# Autodesk Inventor assembly: Shooter
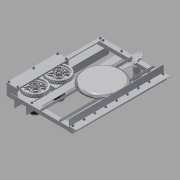
[picture p0: Inventor's stored thumbnail of the model, 180x180]
Saved by Autodesk Inventor 2013 (Build 170138000, 138)
## iProperties
Created: 2013-01-27
Part Number: Shooter
Document SubType Name: Assembly
Designer: Naphat
Author: Naphat
## Documents named in this file (22)
- C:\Autodesk\gruntmaster6000-cad\Shooter6000-cad\Shooter\Shooter.iam
- C:\Autodesk\gruntmaster6000-cad\Shooter6000-cad\Shooter\Basic Wheel\Shooter Basic Design.iam
- C:\Autodesk\gruntmaster6000-cad\Shooter6000-cad\Shooter\26in Angle Channel.ipt
- C:\Autodesk\gruntmaster6000-cad\Shooter6000-cad\Shooter\26in mini C-Channel (rail).ipt
- C:\Autodesk\gruntmaster6000-cad\Shooter6000-cad\Shooter\26in C-Channel (TopPlate Supports).ipt
- C:\Autodesk\gruntmaster6000-cad\Shooter6000-cad\Shooter\3in C-Channel (TopPlate Supports).ipt
- C:\Autodesk\gruntmaster6000-cad\Shooter6000-cad\Shooter\Top Plate.ipt
- C:\Users\Naphat\Documents\Inventor\Content Center Files\R2013\en-US\ANSI B18.3(05)\ANSI B18.3 - 1_4-20 UNC - 1(31).ipt
- C:\Users\Naphat\Documents\Inventor\Content Center Files\R2013\en-US\ASTM F436(1)\ASTM F436 - 1_4(1).ipt
- C:\Users\Naphat\Documents\Inventor\Content Center Files\R2013\en-US\IFI 100 107(2)\IFI 100_107 - 1_4 - 20 Metal Type.ipt
- C:\Autodesk\gruntmaster6000-cad\Shooter6000-cad\Shooter\18in C-Channel Front.ipt
- C:\Autodesk\gruntmaster6000-cad\Shooter6000-cad\Shooter\18in C-Channel Rear.ipt
- C:\Users\Naphat\Documents\Inventor\Content Center Files\R2013\en-US\ANSI B18.3(05)\ANSI B18.3 - 1_4-20 UNC - 1.75(31).ipt
- C:\Autodesk\gruntmaster6000-cad\Shooter6000-cad\Shooter\26in Angle Channel CIM Mount Left.ipt
- C:\Autodesk\gruntmaster6000-cad\Shooter6000-cad\Shooter\26in Angle Channel CIM Mount Right.ipt
- C:\Autodesk\gruntmaster6000-cad\Shooter6000-cad\Shooter\26in C-Channel Left.ipt
- C:\Autodesk\gruntmaster6000-cad\Shooter6000-cad\Shooter\26in C-Channel Right.ipt
- C:\Autodesk\gruntmaster6000-cad\Shooter6000-cad\Shooter\3in C-Channel (TopPlate Supports Rear).ipt
- C:\Autodesk\gruntmaster6000-cad\Shooter6000-cad\Shooter\Motors\CIM Case\CIM Mount Bolt.ipt
- C:\Autodesk\gruntmaster6000-cad\Shooter6000-cad\Shooter\Firing Pin\Firing Pin.iam
- C:\Autodesk\gruntmaster6000-cad\Shooter6000-cad\Shooter\Frisbee.ipt
- C:\Autodesk\gruntmaster6000-cad\Shooter6000-cad\Imported Components\PG27\PG27.ipt
## Components (98 placed, 21 different names)
1. Shooter Basic Design:1 [sub-assembly] — Flush:7, Mate:11, Mate:13, Mate:16, Flush:10, Mate:19, Mate:188
2. Shooter Basic Design:2 [sub-assembly] — Flush:7, Mate:15, Mate:16, Flush:10, Mate:17, Mate:187
3. 26in C-Channel Right:1 — Flush:3, Mate:1, Mate:2, Mate:5, Mate:7, Flush:5, Mate:27, Flush:15, Mate:104, Mate:107, Flush:19, Mate:149, Mate:156, Mate:157, Mate:158
4. 18in C-Channel Rear — Flush:3, Mate:1, Mate:2, Flush:4, Mate:3, Mate:4, Flush:9, Mate:18, Flush:11, Mate:82, Mate:92, Mate:93, Mate:105, Mate:106, Mate:108, Mate:109, Mate:207, Mate:208, Mate:212
5. 18in C-Channel Front — Mate:5, Mate:6, Mate:7, Flush:5, Mate:13, Mate:20, Flush:12, Mate:23, Flush:13, Mate:24, Flush:14, Mate:74, Mate:98, Mate:99, Mate:123, Mate:124, Mate:126, Mate:127, Mate:129, Mate:138
6. 26in C-Channel Left:1 — Flush:4, Mate:3, Mate:4, Mate:6, Mate:8, Mate:9, Mate:75, Mate:76, Mate:77, Mate:78, Mate:79, Mate:80, Mate:81
7. 26in Angle Channel:1 — Mate:8, Mate:9, Flush:9, Mate:11, Mate:15, Mate:25, Mate:36, Mate:38, Mate:39, Mate:40, Mate:41, Mate:42, Mate:43, Mate:44, Mate:45, Mate:46, Mate:47, Mate:48, Mate:49, Mate:50, Mate:51, Mate:52, Mate:53, Mate:54, Mate:55, Mate:56, Mate:57, Mate:58, Mate:59, Mate:60, Mate:61, Mate:62, Mate:63
8. 26in Angle Channel CIM Mount Right:1 — Mate:17, Mate:18, Flush:11, Mate:117, Mate:118, Mate:134, Mate:137, Mate:187, Mate:188, Mate:189, Mate:190, Mate:191, Mate:192, Mate:193, Mate:194, Mate:195, Mate:196
9. 26in Angle Channel CIM Mount Left:3 — Mate:19, Mate:20, Flush:12, Mate:96, Mate:102, Mate:116, Mate:140
10. 26in mini C-Channel (rail):1 — Mate:23, Flush:13, Mate:26, Mate:206
11. 26in mini C-Channel (rail):2 — Mate:24, Flush:14, Mate:25, Mate:26
12. 26in C-Channel (TopPlate Supports):1 — Mate:27, Flush:15, Mate:28, Mate:29, Mate:30, Mate:31, Mate:33, Mate:34, Flush:19, Mate:125, Mate:144, Mate:145, Mate:146, Mate:147, Mate:148, Mate:180, Mate:181, Mate:201, Mate:203
13. 3in C-Channel (TopPlate Supports):1 — Mate:28, Mate:29, Mate:30, Flush:17, Mate:35, Flush:18, Mate:162, Mate:179
14. 3in C-Channel (TopPlate Supports Rear):1 — Mate:31, Mate:33, Mate:34, Mate:182
15. Top Plate:1 — Flush:17, Mate:35, Flush:18, Mate:163, Mate:164, Mate:165, Mate:166, Mate:167, Mate:168, Mate:169, Mate:170, Mate:197, Mate:198, Mate:199
16. CIM Mount Bolt:1 — Mate:192, Mate:196
17. CIM Mount Bolt:2 — Mate:191, Mate:195
18. CIM Mount Bolt:3 — Mate:189, Mate:193
19. CIM Mount Bolt:4 — Mate:190, Mate:194
20. Firing Pin:1 [sub-assembly] — Mate:207, Mate:208, Mate:210, Mate:211
21. Frisbee:1 — Mate:206
22. PG27:1 — Mate:210, Mate:211, Mate:212
23. Hexagon Socket Head Cap Screw - Inch 1/4 - 20 UNC - 1:1 — Mate:36, Mate:72, Mate:91
24. Hexagon Socket Head Cap Screw - Inch 1/4 - 20 UNC - 1:3 — Mate:39, Mate:70, Mate:89
25. Hexagon Socket Head Cap Screw - Inch 1/4 - 20 UNC - 1:4 — Mate:38, Mate:71, Mate:90
26. Hexagon Socket Head Cap Screw - Inch 1/4 - 20 UNC - 1:6 — Mate:199, Mate:200, Mate:202, Mate:204
27. Hexagon Socket Head Cap Screw - Inch 1/4 - 20 UNC - 1:9 — Mate:151, Mate:154, Mate:160
28. Hexagon Socket Head Cap Screw - Inch 1/4 - 20 UNC - 1:10 — Mate:43, Mate:66, Mate:85
29. Hexagon Socket Head Cap Screw - Inch 1/4 - 20 UNC - 1:11 — Mate:40, Mate:69, Mate:88
30. Hexagon Socket Head Cap Screw - Inch 1/4 - 20 UNC - 1:12 — Mate:163, Mate:171, Mate:177, Mate:186
31. Hexagon Socket Head Cap Screw - Inch 1/4 - 20 UNC - 1:14 — Mate:42, Mate:67, Mate:86
32. Hexagon Socket Head Cap Screw - Inch 1/4 - 20 UNC - 1:15 — Mate:173, Mate:176, Mate:184
33. Hexagon Socket Head Cap Screw - Inch 1/4 - 20 UNC - 1:16 — Mate:44, Mate:65, Mate:84
34. Hexagon Socket Head Cap Screw - Inch 1/4 - 20 UNC - 1:17 — Mate:150, Mate:153, Mate:159
35. Hexagon Socket Head Cap Screw - Inch 1/4 - 20 UNC - 1:18 — Mate:45, Mate:64, Mate:83
36. Hexagon Socket Head Cap Screw - Inch 1/4 - 20 UNC - 1:19 — Mate:174, Mate:175, Mate:183
37. Hexagon Socket Head Cap Screw - Inch 1/4 - 20 UNC - 1:22 — Mate:41, Mate:68, Mate:87
38. Hexagon Socket Head Cap Screw - Inch 1/4 - 20 UNC - 1:23 — Mate:152, Mate:155, Mate:161
39. Hexagon Socket Head Cap Screw - Inch 1/4 - 20 UNC - 1:24 — Mate:172, Mate:178, Mate:185
40. Prevailing Torque Type Hex Nut - Inch (IFI) 1/4 - 20 Metal Type:1 — Mate:117, Mate:120
41. Prevailing Torque Type Hex Nut - Inch (IFI) 1/4 - 20 Metal Type:2 — Mate:78, Mate:87
42. Prevailing Torque Type Hex Nut - Inch (IFI) 1/4 - 20 Metal Type:3 — Mate:180, Mate:185
43. Prevailing Torque Type Hex Nut - Inch (IFI) 1/4 - 20 Metal Type:4 — Mate:102, Mate:103
44. Prevailing Torque Type Hex Nut - Inch (IFI) 1/4 - 20 Metal Type:5 — Mate:179, Mate:186
45. Prevailing Torque Type Hex Nut - Inch (IFI) 1/4 - 20 Metal Type:8 — Mate:80, Mate:85
46. Prevailing Torque Type Hex Nut - Inch (IFI) 1/4 - 20 Metal Type:9 — Mate:77, Mate:88
47. Prevailing Torque Type Hex Nut - Inch (IFI) 1/4 - 20 Metal Type:11 — Mate:118, Mate:121
48. Prevailing Torque Type Hex Nut - Inch (IFI) 1/4 - 20 Metal Type:14 — Mate:82, Mate:83
49. Prevailing Torque Type Hex Nut - Inch (IFI) 1/4 - 20 Metal Type:19 — Mate:116, Mate:119
50. Prevailing Torque Type Hex Nut - Inch (IFI) 1/4 - 20 Metal Type:22 — Mate:96, Mate:97
51. Prevailing Torque Type Hex Nut - Inch (IFI) 1/4 - 20 Metal Type:24 — Mate:81, Mate:84
52. Prevailing Torque Type Hex Nut - Inch (IFI) 1/4 - 20 Metal Type:27 — Mate:156, Mate:161
53. Prevailing Torque Type Hex Nut - Inch (IFI) 1/4 - 20 Metal Type:31 — Mate:157, Mate:160
54. Prevailing Torque Type Hex Nut - Inch (IFI) 1/4 - 20 Metal Type:39 — Mate:134, Mate:142
55. Prevailing Torque Type Hex Nut - Inch (IFI) 1/4 - 20 Metal Type:40 — Mate:182, Mate:183
56. Prevailing Torque Type Hex Nut - Inch (IFI) 1/4 - 20 Metal Type:41 — Mate:75, Mate:90
57. Prevailing Torque Type Hex Nut - Inch (IFI) 1/4 - 20 Metal Type:42 — Mate:76, Mate:89
58. Prevailing Torque Type Hex Nut - Inch (IFI) 1/4 - 20 Metal Type:43 — Mate:74, Mate:91
59. Prevailing Torque Type Hex Nut - Inch (IFI) 1/4 - 20 Metal Type:44 — Mate:181, Mate:184
60. Prevailing Torque Type Hex Nut - Inch (IFI) 1/4 - 20 Metal Type:45 — Mate:140, Mate:143
61. Prevailing Torque Type Hex Nut - Inch (IFI) 1/4 - 20 Metal Type:46 — Mate:137, Mate:141
62. Prevailing Torque Type Hex Nut - Inch (IFI) 1/4 - 20 Metal Type:48 — Mate:79, Mate:86
63. Prevailing Torque Type Hex Nut - Inch (IFI) 1/4 - 20 Metal Type:49 — Mate:203, Mate:204
64. Prevailing Torque Type Hex Nut - Inch (IFI) 1/4 - 20 Metal Type:52 — Mate:158, Mate:159
65. Circular Washer (Inch) 1/4:1 — Mate:48, Mate:57, Mate:70
66. Circular Washer (Inch) 1/4:2 — Mate:49, Mate:58, Mate:69
67. Circular Washer (Inch) 1/4:3 — Mate:47, Mate:56, Mate:71
68. Circular Washer (Inch) 1/4:4 — Mate:46, Mate:55, Mate:72
69. Circular Washer (Inch) 1/4:5 — Mate:98, Mate:99, Mate:100, Mate:101
70. Circular Washer (Inch) 1/4:6 — Mate:92, Mate:93, Mate:94, Mate:95
71. Circular Washer (Inch) 1/4:7 — Mate:52, Mate:61, Mate:66
72. Circular Washer (Inch) 1/4:8 — Mate:54, Mate:63, Mate:64
73. Circular Washer (Inch) 1/4:9 — Mate:51, Mate:60, Mate:67
74. Circular Washer (Inch) 1/4:10 — Mate:53, Mate:62, Mate:65
75. Circular Washer (Inch) 1/4:11 — Mate:146, Mate:147, Mate:150, Mate:153
76. Circular Washer (Inch) 1/4:12 — Mate:167, Mate:168, Mate:173, Mate:176
77. Circular Washer (Inch) 1/4:13 — Mate:166, Mate:169, Mate:174, Mate:175
78. Circular Washer (Inch) 1/4:14 — Mate:104, Mate:107, Mate:111, Mate:115
79. Circular Washer (Inch) 1/4:15 — Mate:105, Mate:108, Mate:112, Mate:114
80. Circular Washer (Inch) 1/4:16 — Mate:144, Mate:148, Mate:151, Mate:154
81. Circular Washer (Inch) 1/4:17 — Mate:201, Mate:202
82. Circular Washer (Inch) 1/4:18 — Mate:165, Mate:170, Mate:172, Mate:178
83. Circular Washer (Inch) 1/4:19 — Mate:106, Mate:109, Mate:110, Mate:113
84. Circular Washer (Inch) 1/4:20 — Mate:145, Mate:149, Mate:152, Mate:155
85. Circular Washer (Inch) 1/4:21 — Mate:197, Mate:198, Mate:200
86. Circular Washer (Inch) 1/4:22 — Mate:164, Mate:171, Mate:177
87. Circular Washer (Inch) 1/4:24 — Mate:123, Mate:126, Mate:132
88. Circular Washer (Inch) 1/4:25 — Mate:125, Mate:135, Mate:136, Mate:162
89. Circular Washer (Inch) 1/4:27 — Mate:124, Mate:127, Mate:139
90. Circular Washer (Inch) 1/4:28 — Mate:50, Mate:59, Mate:68
91. Hexagon Socket Head Cap Screw - Inch 1/4 - 20 UNC - 1 3/4:5 — Mate:138, Mate:139, Mate:143
92. Hexagon Socket Head Cap Screw - Inch 1/4 - 20 UNC - 1 3/4:6 — Mate:111, Mate:115, Mate:121
93. Hexagon Socket Head Cap Screw - Inch 1/4 - 20 UNC - 1 3/4:7 — Mate:100, Mate:101, Mate:103
94. Hexagon Socket Head Cap Screw - Inch 1/4 - 20 UNC - 1 3/4:16 — Mate:94, Mate:95, Mate:97
95. Hexagon Socket Head Cap Screw - Inch 1/4 - 20 UNC - 1 3/4:17 — Mate:112, Mate:114, Mate:120
96. Hexagon Socket Head Cap Screw - Inch 1/4 - 20 UNC - 1 3/4:19 — Mate:110, Mate:113, Mate:119
97. Hexagon Socket Head Cap Screw - Inch 1/4 - 20 UNC - 1 3/4:22 — Mate:129, Mate:132, Mate:142
98. Hexagon Socket Head Cap Screw - Inch 1/4 - 20 UNC - 1 3/4:26 — Mate:135, Mate:136, Mate:141
## Relationships (211: Mate 197, Flush 14)
- Flush:3: 26in C-Channel Right:1 ↔ 18in C-Channel Rear
- Mate:1: 26in C-Channel Right:1 ↔ 18in C-Channel Rear
- Mate:2: 26in C-Channel Right:1 ↔ 18in C-Channel Rear
- Flush:4: 18in C-Channel Rear ↔ 26in C-Channel Left:1
- Mate:3: 18in C-Channel Rear ↔ 26in C-Channel Left:1
- Mate:4: 18in C-Channel Rear ↔ 26in C-Channel Left:1
- Mate:5: 26in C-Channel Right:1 ↔ 18in C-Channel Front
- Mate:6: 18in C-Channel Front ↔ 26in C-Channel Left:1
- Mate:7: 26in C-Channel Right:1 ↔ 18in C-Channel Front
- Flush:5: 26in C-Channel Right:1 ↔ 18in C-Channel Front
- Flush:7: Shooter Basic Design:1 ↔ Shooter Basic Design:2
- Mate:8 (-25 mm): 26in C-Channel Left:1 ↔ 26in Angle Channel:1
- Mate:9: 26in C-Channel Left:1 ↔ 26in Angle Channel:1
- Flush:9: 18in C-Channel Rear ↔ 26in Angle Channel:1
- Mate:11 (341.2 mm): Shooter Basic Design:1 ↔ 26in Angle Channel:1
- Mate:13 (-101.6 mm): Shooter Basic Design:1 ↔ 18in C-Channel Front
- Mate:15 (341.2 mm): Shooter Basic Design:2 ↔ 26in Angle Channel:1
- Mate:16 (165.1 mm): Shooter Basic Design:1 ↔ Shooter Basic Design:2
- Flush:10: Shooter Basic Design:1 ↔ Shooter Basic Design:2
- Mate:17: Shooter Basic Design:2 ↔ 26in Angle Channel CIM Mount Right:1
- Mate:18: 18in C-Channel Rear ↔ 26in Angle Channel CIM Mount Right:1
- Flush:11: 18in C-Channel Rear ↔ 26in Angle Channel CIM Mount Right:1
- Mate:19: Shooter Basic Design:1 ↔ 26in Angle Channel CIM Mount Left:3
- Mate:20: 18in C-Channel Front ↔ 26in Angle Channel CIM Mount Left:3
- Flush:12: 18in C-Channel Front ↔ 26in Angle Channel CIM Mount Left:3
- Mate:23: 18in C-Channel Front ↔ 26in mini C-Channel (rail):1
- Flush:13: 18in C-Channel Front ↔ 26in mini C-Channel (rail):1
- Mate:24: 18in C-Channel Front ↔ 26in mini C-Channel (rail):2
- Flush:14: 18in C-Channel Front ↔ 26in mini C-Channel (rail):2
- Mate:25 (69.75 mm): 26in Angle Channel:1 ↔ 26in mini C-Channel (rail):2
- Mate:26 (129.5 mm): 26in mini C-Channel (rail):1 ↔ 26in mini C-Channel (rail):2
- Mate:27: 26in C-Channel Right:1 ↔ 26in C-Channel (TopPlate Supports):1
- Flush:15: 26in C-Channel Right:1 ↔ 26in C-Channel (TopPlate Supports):1
- Mate:28: 26in C-Channel (TopPlate Supports):1 ↔ 3in C-Channel (TopPlate Supports):1
- Mate:29: 26in C-Channel (TopPlate Supports):1 ↔ 3in C-Channel (TopPlate Supports):1
- Mate:30: 26in C-Channel (TopPlate Supports):1 ↔ 3in C-Channel (TopPlate Supports):1
- Mate:31: 26in C-Channel (TopPlate Supports):1 ↔ 3in C-Channel (TopPlate Supports Rear):1
- Mate:33: 26in C-Channel (TopPlate Supports):1 ↔ 3in C-Channel (TopPlate Supports Rear):1
- Mate:34: 26in C-Channel (TopPlate Supports):1 ↔ 3in C-Channel (TopPlate Supports Rear):1
- Flush:17: 3in C-Channel (TopPlate Supports):1 ↔ Top Plate:1
- Mate:35: 3in C-Channel (TopPlate Supports):1 ↔ Top Plate:1
- Flush:18: 3in C-Channel (TopPlate Supports):1 ↔ Top Plate:1
- Mate:36: 26in Angle Channel:1 ↔ Hexagon Socket Head Cap Screw - Inch 1/4 - 20 UNC - 1:1
- Mate:38: 26in Angle Channel:1 ↔ Hexagon Socket Head Cap Screw - Inch 1/4 - 20 UNC - 1:4
- Mate:39: 26in Angle Channel:1 ↔ Hexagon Socket Head Cap Screw - Inch 1/4 - 20 UNC - 1:3
- Mate:40: 26in Angle Channel:1 ↔ Hexagon Socket Head Cap Screw - Inch 1/4 - 20 UNC - 1:11
- Mate:41: 26in Angle Channel:1 ↔ Hexagon Socket Head Cap Screw - Inch 1/4 - 20 UNC - 1:22
- Mate:42: 26in Angle Channel:1 ↔ Hexagon Socket Head Cap Screw - Inch 1/4 - 20 UNC - 1:14
- Mate:43: 26in Angle Channel:1 ↔ Hexagon Socket Head Cap Screw - Inch 1/4 - 20 UNC - 1:10
- Mate:44: 26in Angle Channel:1 ↔ Hexagon Socket Head Cap Screw - Inch 1/4 - 20 UNC - 1:16
- Mate:45: 26in Angle Channel:1 ↔ Hexagon Socket Head Cap Screw - Inch 1/4 - 20 UNC - 1:18
- Mate:46: 26in Angle Channel:1 ↔ Circular Washer (Inch) 1/4:4
- Mate:47: 26in Angle Channel:1 ↔ Circular Washer (Inch) 1/4:3
- Mate:48: 26in Angle Channel:1 ↔ Circular Washer (Inch) 1/4:1
- Mate:49: 26in Angle Channel:1 ↔ Circular Washer (Inch) 1/4:2
- Mate:50: 26in Angle Channel:1 ↔ Circular Washer (Inch) 1/4:28
- Mate:51: 26in Angle Channel:1 ↔ Circular Washer (Inch) 1/4:9
- Mate:52: 26in Angle Channel:1 ↔ Circular Washer (Inch) 1/4:7
- Mate:53: 26in Angle Channel:1 ↔ Circular Washer (Inch) 1/4:10
- Mate:54: 26in Angle Channel:1 ↔ Circular Washer (Inch) 1/4:8
- Mate:55: 26in Angle Channel:1 ↔ Circular Washer (Inch) 1/4:4
- Mate:56: 26in Angle Channel:1 ↔ Circular Washer (Inch) 1/4:3
- Mate:57: 26in Angle Channel:1 ↔ Circular Washer (Inch) 1/4:1
- Mate:58: 26in Angle Channel:1 ↔ Circular Washer (Inch) 1/4:2
- Mate:59: 26in Angle Channel:1 ↔ Circular Washer (Inch) 1/4:28
- Mate:60: 26in Angle Channel:1 ↔ Circular Washer (Inch) 1/4:9
- Mate:61: 26in Angle Channel:1 ↔ Circular Washer (Inch) 1/4:7
- Mate:62: 26in Angle Channel:1 ↔ Circular Washer (Inch) 1/4:10
- Mate:63: 26in Angle Channel:1 ↔ Circular Washer (Inch) 1/4:8
- Mate:64: Hexagon Socket Head Cap Screw - Inch 1/4 - 20 UNC - 1:18 ↔ Circular Washer (Inch) 1/4:8
- Mate:65: Hexagon Socket Head Cap Screw - Inch 1/4 - 20 UNC - 1:16 ↔ Circular Washer (Inch) 1/4:10
- Mate:66: Hexagon Socket Head Cap Screw - Inch 1/4 - 20 UNC - 1:10 ↔ Circular Washer (Inch) 1/4:7
- Mate:67: Hexagon Socket Head Cap Screw - Inch 1/4 - 20 UNC - 1:14 ↔ Circular Washer (Inch) 1/4:9
- Mate:68: Hexagon Socket Head Cap Screw - Inch 1/4 - 20 UNC - 1:22 ↔ Circular Washer (Inch) 1/4:28
- Mate:69: Hexagon Socket Head Cap Screw - Inch 1/4 - 20 UNC - 1:11 ↔ Circular Washer (Inch) 1/4:2
- Mate:70: Hexagon Socket Head Cap Screw - Inch 1/4 - 20 UNC - 1:3 ↔ Circular Washer (Inch) 1/4:1
- Mate:71: Hexagon Socket Head Cap Screw - Inch 1/4 - 20 UNC - 1:4 ↔ Circular Washer (Inch) 1/4:3
- Mate:72: Hexagon Socket Head Cap Screw - Inch 1/4 - 20 UNC - 1:1 ↔ Circular Washer (Inch) 1/4:4
- Mate:74: 18in C-Channel Front ↔ Prevailing Torque Type Hex Nut - Inch (IFI) 1/4 - 20 Metal Type:43
- Mate:75: 26in C-Channel Left:1 ↔ Prevailing Torque Type Hex Nut - Inch (IFI) 1/4 - 20 Metal Type:41
- Mate:76: 26in C-Channel Left:1 ↔ Prevailing Torque Type Hex Nut - Inch (IFI) 1/4 - 20 Metal Type:42
- Mate:77: 26in C-Channel Left:1 ↔ Prevailing Torque Type Hex Nut - Inch (IFI) 1/4 - 20 Metal Type:9
- Mate:78: 26in C-Channel Left:1 ↔ Prevailing Torque Type Hex Nut - Inch (IFI) 1/4 - 20 Metal Type:2
- Mate:79: 26in C-Channel Left:1 ↔ Prevailing Torque Type Hex Nut - Inch (IFI) 1/4 - 20 Metal Type:48
- Mate:80: 26in C-Channel Left:1 ↔ Prevailing Torque Type Hex Nut - Inch (IFI) 1/4 - 20 Metal Type:8
- Mate:81: 26in C-Channel Left:1 ↔ Prevailing Torque Type Hex Nut - Inch (IFI) 1/4 - 20 Metal Type:24
- Mate:82: 18in C-Channel Rear ↔ Prevailing Torque Type Hex Nut - Inch (IFI) 1/4 - 20 Metal Type:14
- Mate:83: Hexagon Socket Head Cap Screw - Inch 1/4 - 20 UNC - 1:18 ↔ Prevailing Torque Type Hex Nut - Inch (IFI) 1/4 - 20 Metal Type:14
- Mate:84: Hexagon Socket Head Cap Screw - Inch 1/4 - 20 UNC - 1:16 ↔ Prevailing Torque Type Hex Nut - Inch (IFI) 1/4 - 20 Metal Type:24
- Mate:85: Hexagon Socket Head Cap Screw - Inch 1/4 - 20 UNC - 1:10 ↔ Prevailing Torque Type Hex Nut - Inch (IFI) 1/4 - 20 Metal Type:8
- Mate:86: Hexagon Socket Head Cap Screw - Inch 1/4 - 20 UNC - 1:14 ↔ Prevailing Torque Type Hex Nut - Inch (IFI) 1/4 - 20 Metal Type:48
- Mate:87: Hexagon Socket Head Cap Screw - Inch 1/4 - 20 UNC - 1:22 ↔ Prevailing Torque Type Hex Nut - Inch (IFI) 1/4 - 20 Metal Type:2
- Mate:88: Hexagon Socket Head Cap Screw - Inch 1/4 - 20 UNC - 1:11 ↔ Prevailing Torque Type Hex Nut - Inch (IFI) 1/4 - 20 Metal Type:9
- Mate:89: Hexagon Socket Head Cap Screw - Inch 1/4 - 20 UNC - 1:3 ↔ Prevailing Torque Type Hex Nut - Inch (IFI) 1/4 - 20 Metal Type:42
- Mate:90: Hexagon Socket Head Cap Screw - Inch 1/4 - 20 UNC - 1:4 ↔ Prevailing Torque Type Hex Nut - Inch (IFI) 1/4 - 20 Metal Type:41
- Mate:91: Hexagon Socket Head Cap Screw - Inch 1/4 - 20 UNC - 1:1 ↔ Prevailing Torque Type Hex Nut - Inch (IFI) 1/4 - 20 Metal Type:43
- Mate:92: 18in C-Channel Rear ↔ Circular Washer (Inch) 1/4:6
- Mate:93: 18in C-Channel Rear ↔ Circular Washer (Inch) 1/4:6
- Mate:94: Circular Washer (Inch) 1/4:6 ↔ Hexagon Socket Head Cap Screw - Inch 1/4 - 20 UNC - 1 3/4:16
- Mate:95: Circular Washer (Inch) 1/4:6 ↔ Hexagon Socket Head Cap Screw - Inch 1/4 - 20 UNC - 1 3/4:16
- Mate:96: 26in Angle Channel CIM Mount Left:3 ↔ Prevailing Torque Type Hex Nut - Inch (IFI) 1/4 - 20 Metal Type:22
- Mate:97: Prevailing Torque Type Hex Nut - Inch (IFI) 1/4 - 20 Metal Type:22 ↔ Hexagon Socket Head Cap Screw - Inch 1/4 - 20 UNC - 1 3/4:16
- Mate:98: 18in C-Channel Front ↔ Circular Washer (Inch) 1/4:5
- Mate:99: 18in C-Channel Front ↔ Circular Washer (Inch) 1/4:5
- Mate:100: Circular Washer (Inch) 1/4:5 ↔ Hexagon Socket Head Cap Screw - Inch 1/4 - 20 UNC - 1 3/4:7
- Mate:101: Circular Washer (Inch) 1/4:5 ↔ Hexagon Socket Head Cap Screw - Inch 1/4 - 20 UNC - 1 3/4:7
- Mate:102: 26in Angle Channel CIM Mount Left:3 ↔ Prevailing Torque Type Hex Nut - Inch (IFI) 1/4 - 20 Metal Type:4
- Mate:103: Prevailing Torque Type Hex Nut - Inch (IFI) 1/4 - 20 Metal Type:4 ↔ Hexagon Socket Head Cap Screw - Inch 1/4 - 20 UNC - 1 3/4:7
- Mate:104: 26in C-Channel Right:1 ↔ Circular Washer (Inch) 1/4:14
- Mate:105: 18in C-Channel Rear ↔ Circular Washer (Inch) 1/4:15
- Mate:106: 18in C-Channel Rear ↔ Circular Washer (Inch) 1/4:19
- Mate:107: 26in C-Channel Right:1 ↔ Circular Washer (Inch) 1/4:14
- Mate:108: 18in C-Channel Rear ↔ Circular Washer (Inch) 1/4:15
- Mate:109: 18in C-Channel Rear ↔ Circular Washer (Inch) 1/4:19
- Mate:110: Circular Washer (Inch) 1/4:19 ↔ Hexagon Socket Head Cap Screw - Inch 1/4 - 20 UNC - 1 3/4:19
- Mate:111: Circular Washer (Inch) 1/4:14 ↔ Hexagon Socket Head Cap Screw - Inch 1/4 - 20 UNC - 1 3/4:6
- Mate:112: Circular Washer (Inch) 1/4:15 ↔ Hexagon Socket Head Cap Screw - Inch 1/4 - 20 UNC - 1 3/4:17
- Mate:113: Circular Washer (Inch) 1/4:19 ↔ Hexagon Socket Head Cap Screw - Inch 1/4 - 20 UNC - 1 3/4:19
- Mate:114: Circular Washer (Inch) 1/4:15 ↔ Hexagon Socket Head Cap Screw - Inch 1/4 - 20 UNC - 1 3/4:17
- Mate:115: Circular Washer (Inch) 1/4:14 ↔ Hexagon Socket Head Cap Screw - Inch 1/4 - 20 UNC - 1 3/4:6
- Mate:116: 26in Angle Channel CIM Mount Left:3 ↔ Prevailing Torque Type Hex Nut - Inch (IFI) 1/4 - 20 Metal Type:19
- Mate:117: 26in Angle Channel CIM Mount Right:1 ↔ Prevailing Torque Type Hex Nut - Inch (IFI) 1/4 - 20 Metal Type:1
- Mate:118: 26in Angle Channel CIM Mount Right:1 ↔ Prevailing Torque Type Hex Nut - Inch (IFI) 1/4 - 20 Metal Type:11
- Mate:119: Prevailing Torque Type Hex Nut - Inch (IFI) 1/4 - 20 Metal Type:19 ↔ Hexagon Socket Head Cap Screw - Inch 1/4 - 20 UNC - 1 3/4:19
- Mate:120: Prevailing Torque Type Hex Nut - Inch (IFI) 1/4 - 20 Metal Type:1 ↔ Hexagon Socket Head Cap Screw - Inch 1/4 - 20 UNC - 1 3/4:17
- Mate:121: Prevailing Torque Type Hex Nut - Inch (IFI) 1/4 - 20 Metal Type:11 ↔ Hexagon Socket Head Cap Screw - Inch 1/4 - 20 UNC - 1 3/4:6
- Flush:19: 26in C-Channel Right:1 ↔ 26in C-Channel (TopPlate Supports):1
- Mate:123: 18in C-Channel Front ↔ Circular Washer (Inch) 1/4:24
- Mate:124: 18in C-Channel Front ↔ Circular Washer (Inch) 1/4:27
- Mate:125: 26in C-Channel (TopPlate Supports):1 ↔ Circular Washer (Inch) 1/4:25
- Mate:126: 18in C-Channel Front ↔ Circular Washer (Inch) 1/4:24
- Mate:127: 18in C-Channel Front ↔ Circular Washer (Inch) 1/4:27
- Mate:129: 18in C-Channel Front ↔ Hexagon Socket Head Cap Screw - Inch 1/4 - 20 UNC - 1 3/4:22
- Mate:132: Circular Washer (Inch) 1/4:24 ↔ Hexagon Socket Head Cap Screw - Inch 1/4 - 20 UNC - 1 3/4:22
- Mate:134: 26in Angle Channel CIM Mount Right:1 ↔ Prevailing Torque Type Hex Nut - Inch (IFI) 1/4 - 20 Metal Type:39
- Mate:135: Circular Washer (Inch) 1/4:25 ↔ Hexagon Socket Head Cap Screw - Inch 1/4 - 20 UNC - 1 3/4:26
- Mate:136: Circular Washer (Inch) 1/4:25 ↔ Hexagon Socket Head Cap Screw - Inch 1/4 - 20 UNC - 1 3/4:26
- Mate:137: 26in Angle Channel CIM Mount Right:1 ↔ Prevailing Torque Type Hex Nut - Inch (IFI) 1/4 - 20 Metal Type:46
- Mate:138: 18in C-Channel Front ↔ Hexagon Socket Head Cap Screw - Inch 1/4 - 20 UNC - 1 3/4:5
- Mate:139: Circular Washer (Inch) 1/4:27 ↔ Hexagon Socket Head Cap Screw - Inch 1/4 - 20 UNC - 1 3/4:5
- Mate:140: 26in Angle Channel CIM Mount Left:3 ↔ Prevailing Torque Type Hex Nut - Inch (IFI) 1/4 - 20 Metal Type:45
- Mate:141: Prevailing Torque Type Hex Nut - Inch (IFI) 1/4 - 20 Metal Type:46 ↔ Hexagon Socket Head Cap Screw - Inch 1/4 - 20 UNC - 1 3/4:26
- Mate:142: Prevailing Torque Type Hex Nut - Inch (IFI) 1/4 - 20 Metal Type:39 ↔ Hexagon Socket Head Cap Screw - Inch 1/4 - 20 UNC - 1 3/4:22
- Mate:143: Prevailing Torque Type Hex Nut - Inch (IFI) 1/4 - 20 Metal Type:45 ↔ Hexagon Socket Head Cap Screw - Inch 1/4 - 20 UNC - 1 3/4:5
- Mate:144: 26in C-Channel (TopPlate Supports):1 ↔ Circular Washer (Inch) 1/4:16
- Mate:145: 26in C-Channel (TopPlate Supports):1 ↔ Circular Washer (Inch) 1/4:20
- Mate:146: 26in C-Channel (TopPlate Supports):1 ↔ Circular Washer (Inch) 1/4:11
- Mate:147: 26in C-Channel (TopPlate Supports):1 ↔ Circular Washer (Inch) 1/4:11
- Mate:148: 26in C-Channel (TopPlate Supports):1 ↔ Circular Washer (Inch) 1/4:16
- Mate:149: 26in C-Channel Right:1 ↔ Circular Washer (Inch) 1/4:20
- Mate:150: Hexagon Socket Head Cap Screw - Inch 1/4 - 20 UNC - 1:17 ↔ Circular Washer (Inch) 1/4:11
- Mate:151: Hexagon Socket Head Cap Screw - Inch 1/4 - 20 UNC - 1:9 ↔ Circular Washer (Inch) 1/4:16
- Mate:152: Hexagon Socket Head Cap Screw - Inch 1/4 - 20 UNC - 1:23 ↔ Circular Washer (Inch) 1/4:20
- Mate:153: Hexagon Socket Head Cap Screw - Inch 1/4 - 20 UNC - 1:17 ↔ Circular Washer (Inch) 1/4:11
- Mate:154: Hexagon Socket Head Cap Screw - Inch 1/4 - 20 UNC - 1:9 ↔ Circular Washer (Inch) 1/4:16
- Mate:155: Hexagon Socket Head Cap Screw - Inch 1/4 - 20 UNC - 1:23 ↔ Circular Washer (Inch) 1/4:20
- Mate:156: 26in C-Channel Right:1 ↔ Prevailing Torque Type Hex Nut - Inch (IFI) 1/4 - 20 Metal Type:27
- Mate:157: 26in C-Channel Right:1 ↔ Prevailing Torque Type Hex Nut - Inch (IFI) 1/4 - 20 Metal Type:31
- Mate:158: 26in C-Channel Right:1 ↔ Prevailing Torque Type Hex Nut - Inch (IFI) 1/4 - 20 Metal Type:52
- Mate:159: Hexagon Socket Head Cap Screw - Inch 1/4 - 20 UNC - 1:17 ↔ Prevailing Torque Type Hex Nut - Inch (IFI) 1/4 - 20 Metal Type:52
- Mate:160: Hexagon Socket Head Cap Screw - Inch 1/4 - 20 UNC - 1:9 ↔ Prevailing Torque Type Hex Nut - Inch (IFI) 1/4 - 20 Metal Type:31
- Mate:161: Hexagon Socket Head Cap Screw - Inch 1/4 - 20 UNC - 1:23 ↔ Prevailing Torque Type Hex Nut - Inch (IFI) 1/4 - 20 Metal Type:27
- Mate:162: 3in C-Channel (TopPlate Supports):1 ↔ Circular Washer (Inch) 1/4:25
- Mate:163: Top Plate:1 ↔ Hexagon Socket Head Cap Screw - Inch 1/4 - 20 UNC - 1:12
- Mate:164: Top Plate:1 ↔ Circular Washer (Inch) 1/4:22
- Mate:165: Top Plate:1 ↔ Circular Washer (Inch) 1/4:18
- Mate:166: Top Plate:1 ↔ Circular Washer (Inch) 1/4:13
- Mate:167: Top Plate:1 ↔ Circular Washer (Inch) 1/4:12
- Mate:168: Top Plate:1 ↔ Circular Washer (Inch) 1/4:12
- Mate:169: Top Plate:1 ↔ Circular Washer (Inch) 1/4:13
- Mate:170: Top Plate:1 ↔ Circular Washer (Inch) 1/4:18
- Mate:171: Hexagon Socket Head Cap Screw - Inch 1/4 - 20 UNC - 1:12 ↔ Circular Washer (Inch) 1/4:22
- Mate:172: Hexagon Socket Head Cap Screw - Inch 1/4 - 20 UNC - 1:24 ↔ Circular Washer (Inch) 1/4:18
- Mate:173: Hexagon Socket Head Cap Screw - Inch 1/4 - 20 UNC - 1:15 ↔ Circular Washer (Inch) 1/4:12
- Mate:174: Hexagon Socket Head Cap Screw - Inch 1/4 - 20 UNC - 1:19 ↔ Circular Washer (Inch) 1/4:13
- Mate:175: Hexagon Socket Head Cap Screw - Inch 1/4 - 20 UNC - 1:19 ↔ Circular Washer (Inch) 1/4:13
- Mate:176: Hexagon Socket Head Cap Screw - Inch 1/4 - 20 UNC - 1:15 ↔ Circular Washer (Inch) 1/4:12
- Mate:177: Hexagon Socket Head Cap Screw - Inch 1/4 - 20 UNC - 1:12 ↔ Circular Washer (Inch) 1/4:22
- Mate:178: Hexagon Socket Head Cap Screw - Inch 1/4 - 20 UNC - 1:24 ↔ Circular Washer (Inch) 1/4:18
- Mate:179: 3in C-Channel (TopPlate Supports):1 ↔ Prevailing Torque Type Hex Nut - Inch (IFI) 1/4 - 20 Metal Type:5
- Mate:180: 26in C-Channel (TopPlate Supports):1 ↔ Prevailing Torque Type Hex Nut - Inch (IFI) 1/4 - 20 Metal Type:3
- Mate:181: 26in C-Channel (TopPlate Supports):1 ↔ Prevailing Torque Type Hex Nut - Inch (IFI) 1/4 - 20 Metal Type:44
- Mate:182: 3in C-Channel (TopPlate Supports Rear):1 ↔ Prevailing Torque Type Hex Nut - Inch (IFI) 1/4 - 20 Metal Type:40
- Mate:183: Hexagon Socket Head Cap Screw - Inch 1/4 - 20 UNC - 1:19 ↔ Prevailing Torque Type Hex Nut - Inch (IFI) 1/4 - 20 Metal Type:40
- Mate:184: Hexagon Socket Head Cap Screw - Inch 1/4 - 20 UNC - 1:15 ↔ Prevailing Torque Type Hex Nut - Inch (IFI) 1/4 - 20 Metal Type:44
- Mate:185: Hexagon Socket Head Cap Screw - Inch 1/4 - 20 UNC - 1:24 ↔ Prevailing Torque Type Hex Nut - Inch (IFI) 1/4 - 20 Metal Type:3
- Mate:186: Hexagon Socket Head Cap Screw - Inch 1/4 - 20 UNC - 1:12 ↔ Prevailing Torque Type Hex Nut - Inch (IFI) 1/4 - 20 Metal Type:5
- Mate:187: Shooter Basic Design:2 ↔ 26in Angle Channel CIM Mount Right:1
- Mate:188: Shooter Basic Design:1 ↔ 26in Angle Channel CIM Mount Right:1
- Mate:189: 26in Angle Channel CIM Mount Right:1 ↔ CIM Mount Bolt:3
- Mate:190: 26in Angle Channel CIM Mount Right:1 ↔ CIM Mount Bolt:4
- Mate:191: 26in Angle Channel CIM Mount Right:1 ↔ CIM Mount Bolt:2
- Mate:192: 26in Angle Channel CIM Mount Right:1 ↔ CIM Mount Bolt:1
- Mate:193: 26in Angle Channel CIM Mount Right:1 ↔ CIM Mount Bolt:3
- Mate:194: 26in Angle Channel CIM Mount Right:1 ↔ CIM Mount Bolt:4
- Mate:195: 26in Angle Channel CIM Mount Right:1 ↔ CIM Mount Bolt:2
- Mate:196: 26in Angle Channel CIM Mount Right:1 ↔ CIM Mount Bolt:1
- Mate:197: Top Plate:1 ↔ Circular Washer (Inch) 1/4:21
- Mate:198: Top Plate:1 ↔ Circular Washer (Inch) 1/4:21
- Mate:199: Top Plate:1 ↔ Hexagon Socket Head Cap Screw - Inch 1/4 - 20 UNC - 1:6
- Mate:200: Hexagon Socket Head Cap Screw - Inch 1/4 - 20 UNC - 1:6 ↔ Circular Washer (Inch) 1/4:21
- Mate:201: 26in C-Channel (TopPlate Supports):1 ↔ Circular Washer (Inch) 1/4:17
- Mate:202: Hexagon Socket Head Cap Screw - Inch 1/4 - 20 UNC - 1:6 ↔ Circular Washer (Inch) 1/4:17
- Mate:203: 26in C-Channel (TopPlate Supports):1 ↔ Prevailing Torque Type Hex Nut - Inch (IFI) 1/4 - 20 Metal Type:49
- Mate:204: Hexagon Socket Head Cap Screw - Inch 1/4 - 20 UNC - 1:6 ↔ Prevailing Torque Type Hex Nut - Inch (IFI) 1/4 - 20 Metal Type:49
- Mate:206: 26in mini C-Channel (rail):1 ↔ Frisbee:1
- Mate:207: 18in C-Channel Rear ↔ Firing Pin:1
- Mate:208: 18in C-Channel Rear ↔ Firing Pin:1
- Mate:210: Firing Pin:1 ↔ PG27:1
- Mate:211: Firing Pin:1 ↔ PG27:1
- Mate:212: 18in C-Channel Rear ↔ PG27:1
